# Autodesk Inventor assembly: Grabber1.1
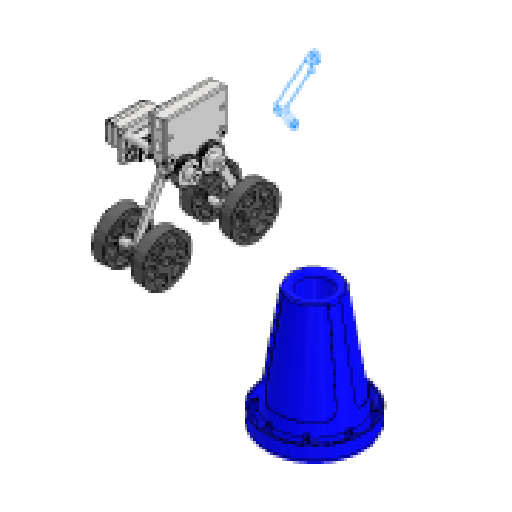
[picture p0: Inventor's stored thumbnail of the model, 512x512]
Saved by Autodesk Inventor 2023 (Build 270158000, 158)
## iProperties
Created: 2022-09-11
Part Number: Grabber1.1
Document SubType Name: Assembly
Designer: deli
Author: deli
## Documents named in this file (20)
- C:\Users\deli\OneDrive - Eastside Preparatory School\FTC\8103-power-play\CAD\Grabber1.1.iam
- C:\Users\deli\OneDrive - Eastside Preparatory School\FTC\8103-power-play\CAD\grabberPlate1.1.ipt
- C:\Users\deli\OneDrive - Eastside Preparatory School\FTC\8103-power-play\CAD\servoPlate1.1.ipt
- C:\Users\deli\OneDrive - Eastside Preparatory School\FTC\8103-power-play\CAD\FTC-parts\goBILDA\2000-0025-0002.ipt
- C:\Users\deli\OneDrive - Eastside Preparatory School\FTC\8103-power-play\CAD\FTC-parts\goBILDA\1308-0016-1006 assembly.ipt
- C:\Users\deli\OneDrive - Eastside Preparatory School\FTC\8103-power-play\CAD\FTC-parts\goBILDA\1611-0514-0006.ipt
- C:\Users\deli\OneDrive - Eastside Preparatory School\FTC\8103-power-play\CAD\FTC-parts\goBILDA\2101-0006-0050 45.2.ipt
- C:\Users\deli\OneDrive - Eastside Preparatory School\FTC\8103-power-play\CAD\FTC-parts\goBILDA\2101-0006-0050 36.7.ipt
- C:\Users\deli\OneDrive - Eastside Preparatory School\FTC\8103-power-play\CAD\FTC-parts\goBILDA\2303-1006-0030 assembly.ipt
- C:\Users\deli\OneDrive - Eastside Preparatory School\FTC\8103-power-play\CAD\FTC-parts\goBILDA\2800-0004-0006.ipt
- C:\Users\deli\OneDrive - Eastside Preparatory School\FTC\8103-power-play\CAD\FTC-parts\goBILDA\2802-0004-0010.ipt
- C:\Users\deli\OneDrive - Eastside Preparatory School\FTC\8103-power-play\CAD\FTC-parts\goBILDA\2802-0004-0022.ipt
- C:\Users\deli\OneDrive - Eastside Preparatory School\FTC\8103-power-play\CAD\FTC-parts\goBILDA\4001-0025-0006 assembly.ipt
- C:\Users\deli\OneDrive - Eastside Preparatory School\FTC\8103-power-play\CAD\FTC-parts\goBILDA\1501-0006-0300.ipt
- C:\Users\deli\OneDrive - Eastside Preparatory School\FTC\8103-power-play\CAD\grabber arm.ipt
- C:\Users\deli\OneDrive - Eastside Preparatory School\FTC\8103-power-play\CAD\FTC-parts\goBILDA\1501-0006-0120.ipt
- C:\Users\deli\OneDrive - Eastside Preparatory School\FTC\8103-power-play\CAD\FTC-parts\goBILDA\1502-0006-0120.ipt
- C:\Users\deli\OneDrive - Eastside Preparatory School\FTC\8103-power-play\CAD\grabber sitck.ipt
- C:\Users\deli\OneDrive - Eastside Preparatory School\FTC\8103-power-play\CAD\FTC-parts\Andymark\am-3572 2IN 8mm Compliant Wheel REV2.ipt
- C:\Users\deli\OneDrive - Eastside Preparatory School\FTC\8103-power-play\CAD\GrabberAdapterToCarbon.ipt
## Components (41 placed, 19 different names)
1. grabberPlate1.1:1 — Mate:97, Flush:2, Flush:3, Mate:138
2. servoPlate1.1:1 — Mate:91, Mate:94
3. 2000-0025-0002:1 — Mate:87, Mate:88
4. 1611-0514-0006:1
5. 1611-0514-0006:2
6. grabberPlate1.1:2 — Mate:96, Mate:136, Flush:4
7. 2101-0006-0050 45.2:1 — Mate:89, Mate:90, Rotation:1
8. 1308-0016-1006 assembly:2 — Mate:133, Mate:134, Mate:135
9. 1308-0016-1006 assembly:3 — Mate:98
10. 2101-0006-0050 36.7:1 — Rotation:1, Mate:137
11. 1611-0514-0006:3 — Mate:137
12. 1611-0514-0006:4
13. 2303-1006-0030 assembly:1
14. 2303-1006-0030 assembly:2
15. 2800-0004-0006:1
16. 2800-0004-0006:2
17. 2800-0004-0006:3
18. 2800-0004-0006:4
19. 2802-0004-0010:1 — Mate:95
20. 2802-0004-0010:2 — Mate:92
21. 2802-0004-0022:1 — Mate:93
22. 2802-0004-0022:2
23. 4001-0025-0006 assembly:1 — Mate:87, Mate:88, Mate:89, Mate:90
24. 1501-0006-0300:1 — Mate:91, Mate:92, Mate:93, Mate:97
25. 1501-0006-0300:2 — Mate:94, Mate:95, Mate:96
26. grabber arm:1 — Mate:98, Mate:100, Mate:102, Mate:105, Mate:106, Mate:109, Mate:112, Mate:117
27. 1501-0006-0120:1 — Mate:100, Mate:102, Mate:114, Mate:115
28. 1502-0006-0120:1 — Mate:105, Mate:106, Mate:107, Mate:108
29. grabber sitck:1
30. am-3572 2IN 8mm Compliant Wheel REV2:1 — Mate:107, Mate:108, Mate:111
31. am-3572 2IN 8mm Compliant Wheel REV2:2 — Mate:114, Mate:115, Mate:116
32. 1502-0006-0120:2 — Mate:109, Mate:111, Mate:117, Mate:118
33. 1501-0006-0120:2 — Mate:112, Mate:116, Mate:118
34. grabber arm:2 — Mate:133, Mate:134, Mate:135
35. 1501-0006-0120:3
36. 1502-0006-0120:3
37. am-3572 2IN 8mm Compliant Wheel REV2:3
38. am-3572 2IN 8mm Compliant Wheel REV2:4
39. 1502-0006-0120:4
40. 1501-0006-0120:4
41. GrabberAdapterToCarbon:1 — Mate:136, Flush:2, Flush:3, Flush:4, Mate:138
## Relationships (91: Mate 82, Angle 4, Flush 4, RelateRotation 1)
- [Mate]: grabberPlate1.1:1 ↔ 1611-0514-0006:2
- [Mate]: grabberPlate1.1:1 ↔ 1611-0514-0006:2
- [Mate]: grabberPlate1.1:1 ↔ 1611-0514-0006:1
- [Mate]: grabberPlate1.1:1 ↔ 1611-0514-0006:1
- [Angle] (180 deg): 2101-0006-0050 45.2:1 ↔ 1308-0016-1006 assembly:2
- [Mate]: 2101-0006-0050 45.2:1 ↔ 1308-0016-1006 assembly:2
- [Flush]: 1611-0514-0006:2 ↔ 2101-0006-0050 36.7:1
- [Mate]: 1611-0514-0006:2 ↔ 2101-0006-0050 36.7:1
- [Angle] (180 deg): 1308-0016-1006 assembly:3 ↔ 2101-0006-0050 36.7:1
- [Mate]: 1308-0016-1006 assembly:3 ↔ 2101-0006-0050 36.7:1
- [Mate]: grabberPlate1.1:2 ↔ 1611-0514-0006:3
- [Mate]: grabberPlate1.1:2 ↔ 1611-0514-0006:4
- [Mate]: grabberPlate1.1:2 ↔ 1611-0514-0006:4
- [Mate]: grabberPlate1.1:2 ↔ 1611-0514-0006:3
- [Mate]: 1611-0514-0006:3 ↔ 2303-1006-0030 assembly:2
- [Mate]: 1611-0514-0006:4 ↔ 2303-1006-0030 assembly:1
- [Mate]: 2101-0006-0050 36.7:1 ↔ 2303-1006-0030 assembly:2
- [Mate]: 2101-0006-0050 45.2:1 ↔ 2303-1006-0030 assembly:1
- [Angle] (180 deg): 2101-0006-0050 36.7:1 ↔ 2303-1006-0030 assembly:2
- [Angle] (180 deg): 2101-0006-0050 45.2:1 ↔ 2303-1006-0030 assembly:1
- [Mate]: servoPlate1.1:1 ↔ 2000-0025-0002:1
- [Mate]: servoPlate1.1:1 ↔ 2000-0025-0002:1
- [Mate]: servoPlate1.1:1 ↔ 2000-0025-0002:1
- [Mate]: 1611-0514-0006:1 ↔ 1308-0016-1006 assembly:2
- [Mate]: 1308-0016-1006 assembly:3 ↔ 1611-0514-0006:3
- [Mate]: 2000-0025-0002:1 ↔ 2800-0004-0006:1
- [Mate]: 2000-0025-0002:1 ↔ 2800-0004-0006:1
- [Mate]: 2000-0025-0002:1 ↔ 2800-0004-0006:2
- [Mate]: 2000-0025-0002:1 ↔ 2800-0004-0006:2
- [Mate]: 2000-0025-0002:1 ↔ 2800-0004-0006:4
- [Mate]: 2000-0025-0002:1 ↔ 2800-0004-0006:4
- [Mate]: 2000-0025-0002:1 ↔ 2800-0004-0006:3
- [Mate]: 2000-0025-0002:1 ↔ 2800-0004-0006:3
- [Mate]: servoPlate1.1:1 ↔ 2802-0004-0010:2
- [Mate]: servoPlate1.1:1 ↔ 2802-0004-0010:1
- [Mate]: servoPlate1.1:1 ↔ 2802-0004-0010:1
- [Mate]: servoPlate1.1:1 ↔ 2802-0004-0010:2
- [Mate]: grabberPlate1.1:2 ↔ 2802-0004-0022:1
- [Mate]: grabberPlate1.1:2 ↔ 2802-0004-0022:2
- [Mate]: grabberPlate1.1:2 ↔ 2802-0004-0022:1
- [Mate]: grabberPlate1.1:2 ↔ 2802-0004-0022:2
- Mate:87: 2000-0025-0002:1 ↔ 4001-0025-0006 assembly:1
- Mate:88: 2000-0025-0002:1 ↔ 4001-0025-0006 assembly:1
- Mate:89: 2101-0006-0050 45.2:1 ↔ 4001-0025-0006 assembly:1
- Mate:90: 2101-0006-0050 45.2:1 ↔ 4001-0025-0006 assembly:1
- Mate:91: servoPlate1.1:1 ↔ 1501-0006-0300:1
- Mate:92: 2802-0004-0010:2 ↔ 1501-0006-0300:1
- Mate:93: 2802-0004-0022:1 ↔ 1501-0006-0300:1
- Mate:94: servoPlate1.1:1 ↔ 1501-0006-0300:2
- Mate:95: 2802-0004-0010:1 ↔ 1501-0006-0300:2
- Mate:96: grabberPlate1.1:2 ↔ 1501-0006-0300:2
- Mate:97: grabberPlate1.1:1 ↔ 1501-0006-0300:1
- Mate:98: 1308-0016-1006 assembly:3 ↔ grabber arm:1
- Mate:100: grabber arm:1 ↔ 1501-0006-0120:1
- Mate:102: grabber arm:1 ↔ 1501-0006-0120:1
- Mate:105: grabber arm:1 ↔ 1502-0006-0120:1
- Mate:106: grabber arm:1 ↔ 1502-0006-0120:1
- Mate:107: 1502-0006-0120:1 ↔ am-3572 2IN 8mm Compliant Wheel REV2:1
- Mate:108: 1502-0006-0120:1 ↔ am-3572 2IN 8mm Compliant Wheel REV2:1
- Mate:109: grabber arm:1 ↔ 1502-0006-0120:2
- Mate:111: am-3572 2IN 8mm Compliant Wheel REV2:1 ↔ 1502-0006-0120:2
- Mate:112: grabber arm:1 ↔ 1501-0006-0120:2
- Mate:114: 1501-0006-0120:1 ↔ am-3572 2IN 8mm Compliant Wheel REV2:2
- Mate:115: 1501-0006-0120:1 ↔ am-3572 2IN 8mm Compliant Wheel REV2:2
- Mate:116: am-3572 2IN 8mm Compliant Wheel REV2:2 ↔ 1501-0006-0120:2
- Mate:117: grabber arm:1 ↔ 1502-0006-0120:2
- Mate:118: 1502-0006-0120:2 ↔ 1501-0006-0120:2
- [Mate]: grabber arm:2 ↔ 1501-0006-0120:3
- [Mate]: grabber arm:2 ↔ 1501-0006-0120:3
- [Mate]: grabber arm:2 ↔ 1502-0006-0120:3
- [Mate]: grabber arm:2 ↔ 1502-0006-0120:3
- [Mate]: 1502-0006-0120:3 ↔ am-3572 2IN 8mm Compliant Wheel REV2:3
- [Mate]: 1502-0006-0120:3 ↔ am-3572 2IN 8mm Compliant Wheel REV2:3
- [Mate]: grabber arm:2 ↔ 1502-0006-0120:4
- [Mate]: am-3572 2IN 8mm Compliant Wheel REV2:3 ↔ 1502-0006-0120:4
- [Mate]: grabber arm:2 ↔ 1501-0006-0120:4
- [Mate]: 1501-0006-0120:3 ↔ am-3572 2IN 8mm Compliant Wheel REV2:4
- [Mate]: 1501-0006-0120:3 ↔ am-3572 2IN 8mm Compliant Wheel REV2:4
- [Mate]: am-3572 2IN 8mm Compliant Wheel REV2:4 ↔ 1501-0006-0120:4
- [Mate]: grabber arm:2 ↔ 1502-0006-0120:4
- [Mate]: 1502-0006-0120:4 ↔ 1501-0006-0120:4
- Mate:133: 1308-0016-1006 assembly:2 ↔ grabber arm:2
- Mate:134: 1308-0016-1006 assembly:2 ↔ grabber arm:2
- Mate:135: 1308-0016-1006 assembly:2 ↔ grabber arm:2
- Rotation:1 [RelateRotation] (1 ul): 2101-0006-0050 45.2:1 ↔ 2101-0006-0050 36.7:1
- Mate:136: grabberPlate1.1:2 ↔ GrabberAdapterToCarbon:1
- Mate:137: 2101-0006-0050 36.7:1 ↔ 1611-0514-0006:3
- Flush:2: grabberPlate1.1:1 ↔ GrabberAdapterToCarbon:1
- Flush:3: grabberPlate1.1:1 ↔ GrabberAdapterToCarbon:1
- Flush:4: grabberPlate1.1:2 ↔ GrabberAdapterToCarbon:1
- Mate:138: grabberPlate1.1:1 ↔ GrabberAdapterToCarbon:1
## Named parameters: d15_d75 = 0 mm, d16_d76 = 0 mm, d17_d77 = 0 mm, d18_d78 = 0 mm, d22_d87 = 180 deg, d23_d88 = 0 mm, d24_d95 = 0 mm, d25_d96 = 0 mm, d26_d97 = 180 deg, d27_d98 = 0 mm, d29_d101 = 0 mm, d30_d102 = 0 mm, d159_d155 = 0 mm, d160_d156 = 0 mm, d161_d157 = 0 mm, d162_d158 = 0 mm, d163_d139 = 0 mm, d164_d141 = 0 mm, d165_d144 = 0 mm, d194_d145 = 0 mm, d195_d147 = 0 mm, d196_d148 = 0 mm, d197_d149 = 0 mm, d198_d151 = 0 mm, d199_d152 = 0 mm, d200_d154 = 0 mm
